# Autodesk Inventor assembly: test
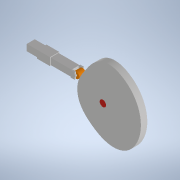
[picture p0: Inventor's stored thumbnail of the model, 180x180]
Saved by Autodesk Inventor 2022 (Build 260153000, 153)
## iProperties
Created: 2023-03-23
Part Number: test
Document SubType Name: Assembly
Designer: JOU
Author: JOU
## Documents named in this file (6)
- C:\Users\JOU\Desktop\git\Special-project\test.iam
- C:\Users\JOU\Desktop\git\Special-project\axis.ipt
- C:\Users\JOU\Desktop\git\Special-project\CamProfile_Trans_offset_roller_Cycloid.ipt
- C:\Users\JOU\Desktop\git\Special-project\axis_rf_fix.ipt
- C:\Users\JOU\Desktop\git\Special-project\axis_rf.ipt
- C:\Users\JOU\Desktop\git\Special-project\rf.ipt
## Components (5 placed, 5 different names)
1. axis:1 — 插入:1
2. CamProfile_Trans_offset_roller_Cycloid:1 — 插入:1, 角度:1, 相切:1
3. axis_rf_fix:1 — 貼合:1, 貼合:2, 貼合:3, 貼合:4, 齊平:1
4. axis_rf:1 — 貼合:1, 貼合:2, 貼合:5, 貼合:6
5. rf:1 — 貼合:5, 貼合:6, 相切:1
## Relationships (10: Mate 6, Insert 1, Flush 1, Angle 1, Tangent 1)
- 插入:1 [Insert]: axis:1 ↔ CamProfile_Trans_offset_roller_Cycloid:1
- 貼合:1 [Mate]: axis_rf_fix:1 ↔ axis_rf:1
- 貼合:2 [Mate]: axis_rf_fix:1 ↔ axis_rf:1
- 貼合:3 [Mate] (6.25 mm): axis_rf_fix:1
- 貼合:4 [Mate] (12 mm): axis_rf_fix:1
- 齊平:1 [Flush] (80 mm): axis_rf_fix:1
- 角度:1 [Angle] (-20 deg): CamProfile_Trans_offset_roller_Cycloid:1
- 貼合:5 [Mate]: axis_rf:1 ↔ rf:1
- 貼合:6 [Mate]: axis_rf:1 ↔ rf:1
- 相切:1 [Tangent]: CamProfile_Trans_offset_roller_Cycloid:1 ↔ rf:1
